# Autodesk Inventor assembly: DelrinX-Wheel-Bottom_MIR3
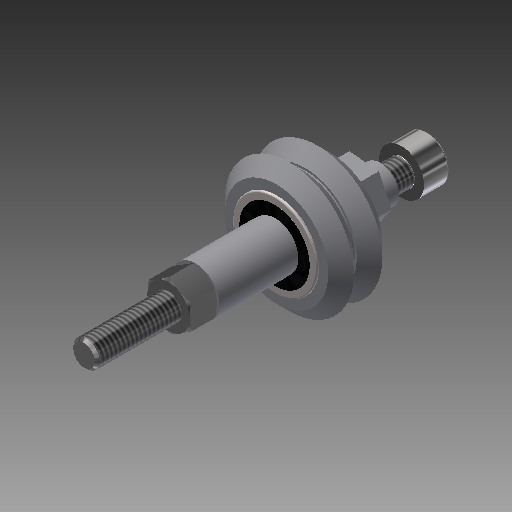
[picture p0: Inventor's stored thumbnail of the model, 512x512]
Saved by Autodesk Inventor 2017 (Build 210142000, 142)
## iProperties
Created: 2016-07-20
Part Number: DelrinX-Wheel-Bottom_MIR3
Document SubType Name: Assembly
Designer: User
Author: User
## Documents named in this file (6)
- C:\All INVENTOR\SL-Inventor\SL-Beast 3D Printer\DelrinX-Wheel-Bottom_MIR3.iam
- C:\All INVENTOR\SL-Inventor\SL-Beast 3D Printer\DelrinWheel_MIR3.iam
- C:\All INVENTOR\SL-Inventor\SL-Beast 3D Printer\Long-Spacer_MIR3.ipt
- C:\All INVENTOR\SL-Inventor\SL-Beast 3D Printer\ANSI B18.3.1M - M5x0.8 x 60NEW_MIR3.ipt
- C:\All INVENTOR\SL-Inventor\SL-Beast 3D Printer\en-US\ANSI B 18.2.4.1 M(1)\ANSI B 18.2.4.1 M - M5 x 0.8Style 2.ipt
- C:\All INVENTOR\SL-Inventor\SL-Beast 3D Printer\Eccentric Spacer_MIR4.ipt
## Components (5 placed, 5 different names)
1. DelrinWheel_MIR3:1 [sub-assembly] — Mate:2, Mate:1, Mate:4
2. Long-Spacer_MIR3:1 — Insert:1
3. ANSI B18.3.1M - M5x0.8 x 60NEW_MIR3:1 — Mate:2, Mate:1, Mate:3
4. Hex Nut Metric M5 x 0.8:1 — Insert:1
5. Eccentric Spacer_MIR4:1 — Mate:4, Mate:3
## Relationships (5: Mate 4, Insert 1)
- Mate:2 (13 mm): DelrinWheel_MIR3:1 ↔ ANSI B18.3.1M - M5x0.8 x 60NEW_MIR3:1
- Mate:1: DelrinWheel_MIR3:1 ↔ ANSI B18.3.1M - M5x0.8 x 60NEW_MIR3:1
- Insert:1: Long-Spacer_MIR3:1 ↔ Hex Nut Metric M5 x 0.8:1
- Mate:4: DelrinWheel_MIR3:1 ↔ Eccentric Spacer_MIR4:1
- Mate:3: ANSI B18.3.1M - M5x0.8 x 60NEW_MIR3:1 ↔ Eccentric Spacer_MIR4:1
